# Autodesk Inventor assembly: sprocket and bevel gear on shaft
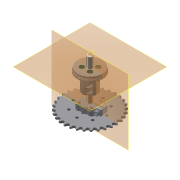
[picture p0: Inventor's stored thumbnail of the model, 180x180]
Saved by Autodesk Inventor 2018 (Build 220112000, 112)
## iProperties
Created: 2019-09-29
Part Number: sprocket and bevel gear on shaft
Document SubType Name: Assembly
Designer: ball
Author: ball
## Documents named in this file (4)
- C:\FTC\FTC8863CAD\2019 Robot\Mecanum Drive Train\sprocket and bevel gear on shaft.iam
- C:\FTC\FTC8863CAD\Actobotics\634 parts\634078.ipt
- C:\FTC\FTC8863CAD\2019 Robot\Mecanum Drive Train\bevel gear with clamping hub.iam
- C:\FTC\FTC8863CAD\2019 Robot\Mecanum Drive Train\32 spocket with hub.iam
## Components (3 placed, 3 different names)
1. 634078:1 — Mate:1, Mate:3, Mate:4, Mate:5, Mate:6, Flush:1, Mate:7, Angle:1
2. bevel gear with clamping hub:1 [sub-assembly] — Mate:4, Mate:5, Mate:6, Flush:1, Flush:2
3. 32 spocket with hub:1 [sub-assembly] — Mate:1, Mate:3
## Relationships (9: Mate 6, Flush 2, Angle 1)
- Mate:1: 634078:1 ↔ 32 spocket with hub:1
- Mate:3 (-25.4 mm): 634078:1 ↔ 32 spocket with hub:1
- Mate:4: 634078:1 ↔ bevel gear with clamping hub:1
- Mate:5: 634078:1 ↔ bevel gear with clamping hub:1
- Mate:6: 634078:1 ↔ bevel gear with clamping hub:1
- Flush:1 (-12.7 mm): 634078:1 ↔ bevel gear with clamping hub:1
- Mate:7: 634078:1
- Angle:1 (90 deg): 634078:1
- Flush:2: bevel gear with clamping hub:1
